# Autodesk Inventor assembly: Assembly1
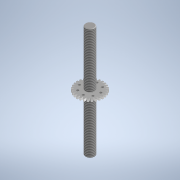
[picture p0: Inventor's stored thumbnail of the model, 180x180]
Saved by Autodesk Inventor 2020 (Build 240168000, 168)
## iProperties
Created: 2020-05-18
Part Number: Assembly1
Document SubType Name: Assembly
Designer: Gebruiker
Author: Gebruiker
## Documents named in this file (3)
- C:\Users\Gebruiker\Documents\GitHub\BeerMinder\3D-model\servo\Assembly1.iam
- C:\Users\Gebruiker\Desktop\SMR\Robotarm\tandwiel1.ipt
- C:\Users\Gebruiker\Desktop\SMR\Robotarm\as.ipt
## Components (2 placed, 2 different names)
1. tandwiel1:1 — Mate:1, Mate:2
2. as:1 — Mate:1, Mate:2
## Relationships (2: Mate 2)
- Mate:1: tandwiel1:1 ↔ as:1
- Mate:2: tandwiel1:1 ↔ as:1
